# Autodesk Inventor assembly: flexMid
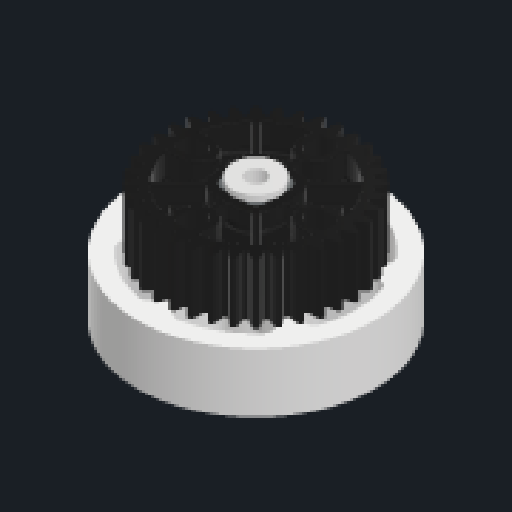
[picture p0: Inventor's stored thumbnail of the model, 512x512]
Saved by Autodesk Inventor 2024.2 (Build 282272000, 272)
## iProperties
Created: 2024-01-28
Part Number: flexMid
Document SubType Name: Assembly
Designer: reima
Mass: 23.8848 g
Surface Area: 189.007 cm^2
Volume: 23.7292 cm^3
Density: 1.00656 g/cm^3
Author: reima
## Documents named in this file (6)
- O:\cad\61002g-cad\subasm\flexMid.iam
- O:\cad\61002g-cad\VEX parts\Motion\Wheels\Flex Wheels\2.000 Flex Wheel\2.000 30A .500.ipt
- O:\cad\61002g-cad\VEX parts\Motion\Wheels\Flex Wheels\2.000 Flex Wheel.ipt
- O:\cad\61002g-cad\VEX parts\Motion\Gears\HS Gear\HS 36T Gear, No Insert.iam
- O:\cad\61002g-cad\VEX parts\Motion\Gears\HS Gear.iam
- O:\cad\61002g-cad\VEX parts\Motion\Insert Circle.ipt
## Components (4 placed, 3 different names)
1. 2.000 30A .500:1 — Insert:1, Insert:3
2. HS 36T Gear, No Insert:1 [sub-assembly] — Insert:1, Insert:2
3. Insert Circle:1 — Insert:2
4. Insert Circle:2 — Insert:3
## Relationships (3: Insert 3)
- Insert:1: 2.000 30A .500:1 ↔ HS 36T Gear, No Insert:1
- Insert:2: HS 36T Gear, No Insert:1 ↔ Insert Circle:1
- Insert:3 (1.5875 mm): 2.000 30A .500:1 ↔ Insert Circle:2
